# Autodesk Inventor assembly: handAssembly
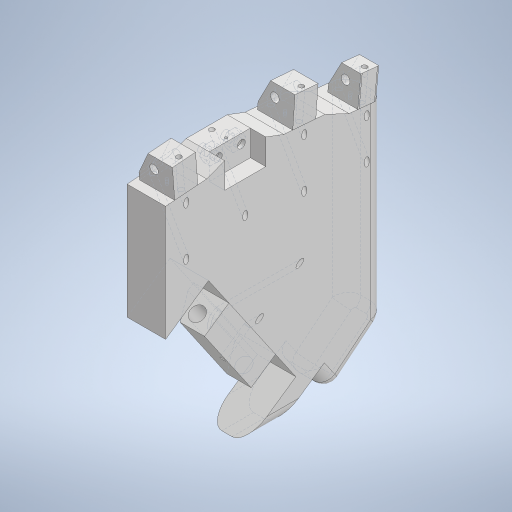
[picture p0: Inventor's stored thumbnail of the model, 512x512]
Saved by Autodesk Inventor 2024 (Build 280153000, 153)
## iProperties
Created: 2024-06-09
Part Number: handAssembly
Document SubType Name: Assembly
Designer: omiye
Author: omiye
## Documents named in this file (5)
- C:\Projects\roboticHand\fingerModels\handAssembly.iam
- C:\Projects\roboticHand\fingerModels\palm.ipt
- C:\Projects\roboticHand\fingerModels\normMale.ipt
- C:\Projects\roboticHand\fingerModels\pinkyMale.ipt
- C:\Projects\roboticHand\fingerModels\thumbConnectors\thumbMale.ipt
## Components (5 placed, 4 different names)
1. palm:1 — Mate:6, Mate:7, Mate:8, Mate:9, Mate:10, Mate:11, Mate:42, Mate:43, Mate:44, Mate:45, Mate:46, Mate:47
2. normMale:2 — Mate:9, Mate:10, Mate:11
3. normMale:4 — Mate:6, Mate:7, Mate:8
4. pinkyMale:1 — Mate:42, Mate:43, Mate:44
5. thumbMale:1 — Mate:45, Mate:46, Mate:47
## Relationships (12: Mate 12)
- Mate:6: palm:1 ↔ normMale:4
- Mate:7: palm:1 ↔ normMale:4
- Mate:8: palm:1 ↔ normMale:4
- Mate:9: palm:1 ↔ normMale:2
- Mate:10: palm:1 ↔ normMale:2
- Mate:11: palm:1 ↔ normMale:2
- Mate:42: palm:1 ↔ pinkyMale:1
- Mate:43: palm:1 ↔ pinkyMale:1
- Mate:44: palm:1 ↔ pinkyMale:1
- Mate:45: palm:1 ↔ thumbMale:1
- Mate:46: palm:1 ↔ thumbMale:1
- Mate:47: palm:1 ↔ thumbMale:1
